# Autodesk Inventor assembly: instrumentBody
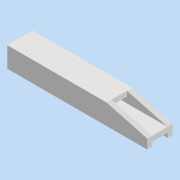
[picture p0: Inventor's stored thumbnail of the model, 180x180]
Saved by Autodesk Inventor 2021 (Build 250183000, 183)
## iProperties
Created: 2021-02-01
Part Number: instrumentBody
Document SubType Name: Assembly
Designer: garre
Author: garre
## Documents named in this file (4)
- C:\Users\garre\Desktop\Parts\instrumentBody.iam
- C:\Users\garre\Desktop\Parts\bodySidePlate.ipt
- C:\Users\garre\Desktop\Parts\bodyTopPlate.ipt
- C:\Users\garre\Desktop\Parts\bodyBotPlate.ipt
## Components (4 placed, 3 different names)
1. bodySidePlate:1 — Mate:2, Flush:3, Flush:4, Mate:4
2. bodySidePlate:2 — Mate:1, Flush:1, Flush:2, Mate:3, Flush:5
3. bodyTopPlate:1 — Mate:1, Flush:1, Flush:2, Mate:2, Flush:3, Flush:4
4. bodyBotPlate:1 — Mate:3, Flush:5, Mate:4
## Relationships (9: Flush 5, Mate 4)
- Mate:1: bodySidePlate:2 ↔ bodyTopPlate:1
- Flush:1: bodySidePlate:2 ↔ bodyTopPlate:1
- Flush:2: bodySidePlate:2 ↔ bodyTopPlate:1
- Mate:2: bodySidePlate:1 ↔ bodyTopPlate:1
- Flush:3: bodySidePlate:1 ↔ bodyTopPlate:1
- Flush:4: bodySidePlate:1 ↔ bodyTopPlate:1
- Mate:3: bodySidePlate:2 ↔ bodyBotPlate:1
- Flush:5: bodySidePlate:2 ↔ bodyBotPlate:1
- Mate:4: bodySidePlate:1 ↔ bodyBotPlate:1
